# Autodesk Inventor assembly: PLS-14
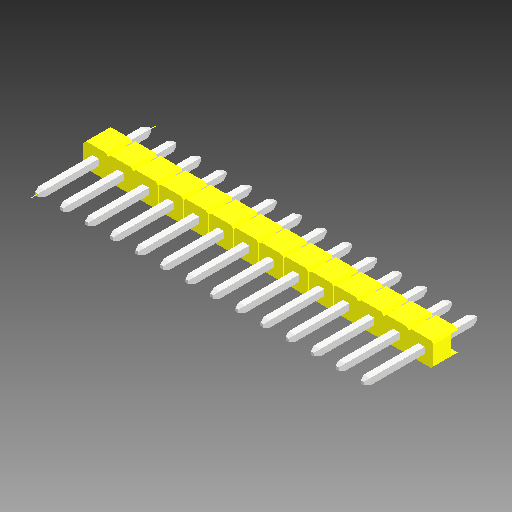
[picture p0: Inventor's stored thumbnail of the model, 512x512]
Saved by Autodesk Inventor 2020 (Build 240168000, 168)
## iProperties
Created: 2024-06-27
Part Number: PLS-14
Description: FreeCAD Model
Document SubType Name: Assembly
Designer: Ivan
Authority: Unknown
Mass: 0.211945 g
Surface Area: 8.76831 cm^2
Volume: 0.211945 cm^3
Density: 1 g/cm^3
Sending System: FreeCAD
Preprocessor: Open CASCADE STEP processor 7.6
Title: Open CASCADE Shape Model
## Documents named in this file (16)
- C:\!projects\DASH-\3D\Dash-V1\step\PLS-14\PLS-14.iam
- C:\!projects\DASH-\3D\Dash-V1\step\PLS-14\Frame.ipt
- C:\!projects\DASH-\3D\Dash-V1\step\PLS-14\Pin01.ipt
- C:\!projects\DASH-\3D\Dash-V1\step\PLS-14\Pin002.ipt
- C:\!projects\DASH-\3D\Dash-V1\step\PLS-14\Pin003.ipt
- C:\!projects\DASH-\3D\Dash-V1\step\PLS-14\Pin004.ipt
- C:\!projects\DASH-\3D\Dash-V1\step\PLS-14\Pin005.ipt
- C:\!projects\DASH-\3D\Dash-V1\step\PLS-14\Pin006.ipt
- C:\!projects\DASH-\3D\Dash-V1\step\PLS-14\Pin007.ipt
- C:\!projects\DASH-\3D\Dash-V1\step\PLS-14\Pin008.ipt
- C:\!projects\DASH-\3D\Dash-V1\step\PLS-14\Pin009.ipt
- C:\!projects\DASH-\3D\Dash-V1\step\PLS-14\Pin010.ipt
- C:\!projects\DASH-\3D\Dash-V1\step\PLS-14\Pin011.ipt
- C:\!projects\DASH-\3D\Dash-V1\step\PLS-14\Pin012.ipt
- C:\!projects\DASH-\3D\Dash-V1\step\PLS-14\Pin013.ipt
- C:\!projects\DASH-\3D\Dash-V1\step\PLS-14\Pin014.ipt
## Components (15 placed, 15 different names)
1. 37
2. 38 — Совмещение:1
3. 39
4. 40
5. 41
6. 42
7. 43
8. 44
9. 45
10. 46
11. 47
12. 48
13. 49
14. 50
15. 51
## Relationships (1: Mate 1)
- Совмещение:1 [Mate]: 38
